# Autodesk Inventor assembly: zlozenieniewiem
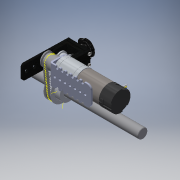
[picture p0: Inventor's stored thumbnail of the model, 180x180]
Saved by Autodesk Inventor 2019 (Build 230136000, 136)
## iProperties
Created: 2020-08-21
Part Number: zlozenieniewiem
Document SubType Name: Assembly
Designer: estee
Author: estee
## Documents named in this file (5)
- C:\Users\estee\OneDrive\Pulpit\projejt\zlozenieniewiem.iam
- C:\Users\estee\OneDrive\Pulpit\projejt\ModulDuzegoKola.iam
- C:\Users\estee\OneDrive\Pulpit\projejt\ModulSilnika.iam
- C:\Users\estee\OneDrive\Pulpit\projejt\PasekZebatyNowy.iam
- C:\Users\estee\OneDrive\Pulpit\projejt\ModulWalkaNapinajacego.iam
## Components (4 placed, 4 different names)
1. ModulDuzegoKola:1 [sub-assembly] — Mate:1, Mate:2
2. ModulSilnika:1 [sub-assembly] — Mate:3, Mate:4
3. PasekZebatyNowy:1 [sub-assembly] — Mate:1, Mate:2, Mate:3, Mate:4, Mate:5, Mate:6
4. ModulWalkaNapinajacego:1 [sub-assembly] — Mate:5, Mate:6
## Relationships (6: Mate 6)
- Mate:1: ModulDuzegoKola:1 ↔ PasekZebatyNowy:1
- Mate:2 (0.5 mm): ModulDuzegoKola:1 ↔ PasekZebatyNowy:1
- Mate:3: ModulSilnika:1 ↔ PasekZebatyNowy:1
- Mate:4 (0.5 mm): ModulSilnika:1 ↔ PasekZebatyNowy:1
- Mate:5: PasekZebatyNowy:1 ↔ ModulWalkaNapinajacego:1
- Mate:6 (0.5 mm): PasekZebatyNowy:1 ↔ ModulWalkaNapinajacego:1
